# Autodesk Inventor assembly: Coil Designs
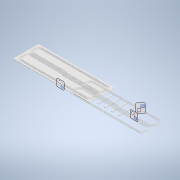
[picture p0: Inventor's stored thumbnail of the model, 180x180]
Saved by Autodesk Inventor 2021 (Build 250183000, 183)
## iProperties
Created: 2022-01-19
Part Number: Coil Designs
Document SubType Name: Assembly
Designer: avan411
Author: avan411
## Documents named in this file (4)
- H:\GitRepos\Coil Designs.iam
- H:\GitRepos\FerriteBar.ipt
- H:\GitRepos\Part2.ipt
- H:\GitRepos\coil.ipt
## Components (20 placed, 3 different names)
1. PrimaryCoilLayer:1 — Mate:5
2. coil:1
3. FerriteBar:2 — Mate:1, Mate:2
4. FerriteBar:1 — Mate:1, Mate:2
5. FerriteBar:3
6. FerriteBar:4
7. FerriteBar:5
8. FerriteBar:6
9. FerriteBar:7
10. FerriteBar:8
11. FerriteBar:9
12. FerriteBar:10
13. FerriteBar:11
14. FerriteBar:12
15. FerriteBar:13
16. FerriteBar:14
17. FerriteBar:15
18. FerriteBar:16
19. FerriteBar:17
20. FerriteBar:18 — Mate:5
## Component patterns: (9 elements, first: FerriteBar:2 + FerriteBar:1)
## Relationships (3: Mate 3)
- Mate:1: FerriteBar:2 ↔ FerriteBar:1
- Mate:2: FerriteBar:2 ↔ FerriteBar:1
- Mate:5 (41.6 mm): PrimaryCoilLayer:1 ↔ FerriteBar:18
